# Autodesk Inventor assembly: drvassembly
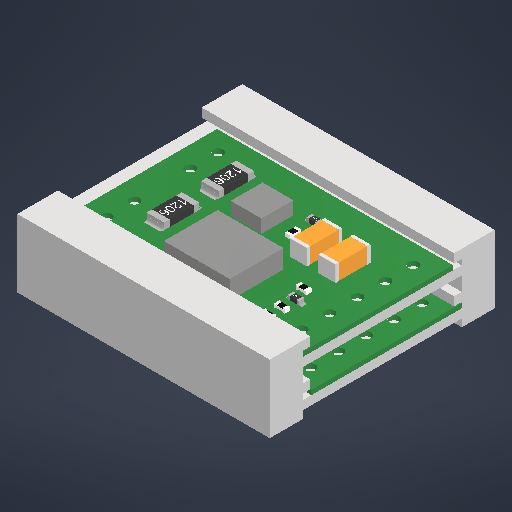
[picture p0: Inventor's stored thumbnail of the model, 512x512]
Saved by Autodesk Inventor 2026.2 (Build 302298010, 298A)
## iProperties
Created: 2026-05-11
Part Number: drvassembly
Document SubType Name: Assembly
Designer: karol
Author: karol
## Documents named in this file (3)
- C:\Users\karol\OneDrive\Desktop\robo\bolt\cad\assembly\drvassembly.iam
- C:\Users\karol\OneDrive\Desktop\robo\bolt\cad\ready parts\drvholder.ipt
- C:\Users\karol\OneDrive\Desktop\robo\bolt\cad\pcbs\drv\drv\drv.iam
## Components (3 placed, 2 different names)
1. drvholder:1 — Mate:1, Mate:2, Mate:3, Mate:4
2. drv:2 [sub-assembly] — Mate:1, Mate:2
3. drv:3 [sub-assembly] — Mate:3, Mate:4
## Relationships (4: Mate 4)
- Mate:1: drvholder:1 ↔ drv:2
- Mate:2: drvholder:1 ↔ drv:2
- Mate:3: drvholder:1 ↔ drv:3
- Mate:4: drvholder:1 ↔ drv:3
